# Autodesk Inventor assembly: DishBoard
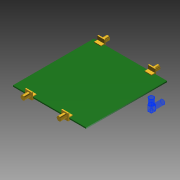
[picture p0: Inventor's stored thumbnail of the model, 180x180]
Saved by Autodesk Inventor 2014 (Build 180170000, 170)
## iProperties
Created: 2015-01-07
Part Number: DishBoard
Document SubType Name: Assembly
Designer: Owner
Author: Owner
## Documents named in this file (5)
- C:\Users\Owner\Documents\APC\FrontEnd\IAM\Dish\DishBoard.iam
- C:\Users\Owner\Documents\APC\FrontEnd\IAM\Dish\Dish_Board.ipt
- C:\Users\Owner\Documents\APC\FrontEnd\IAM\Common\SMA_Edge.ipt
- C:\Users\Owner\Documents\APC\FrontEnd\IAM\Common\SMA_Up.ipt
- C:\Users\Owner\Documents\APC\FrontEnd\IAM\Common\SMA_RightAngle.ipt
## Components (7 placed, 4 different names)
1. Dish_Board:1 — Mate:1, Mate:2, Mate:3, Mate:4, Mate:5, Mate:6, Mate:7, Mate:8, Flush:1, Flush:2, Flush:3, Flush:4, Mate:9
2. SMA_Edge:1 — Mate:5, Mate:7, Flush:1
3. SMA_Edge:2 — Mate:6, Mate:8, Flush:2
4. SMA_Edge:3 — Mate:1, Mate:2, Flush:4
5. SMA_Edge:4 — Mate:3, Mate:4, Flush:3
6. SMA_Up:1 — Mate:9, Mate:10, Mate:11
7. SMA_RightAngle:1 — Mate:10, Mate:11
## Relationships (15: Mate 11, Flush 4)
- Mate:1: Dish_Board:1 ↔ SMA_Edge:3
- Mate:2: Dish_Board:1 ↔ SMA_Edge:3
- Mate:3: Dish_Board:1 ↔ SMA_Edge:4
- Mate:4: Dish_Board:1 ↔ SMA_Edge:4
- Mate:5: Dish_Board:1 ↔ SMA_Edge:1
- Mate:6: Dish_Board:1 ↔ SMA_Edge:2
- Mate:7: Dish_Board:1 ↔ SMA_Edge:1
- Mate:8: Dish_Board:1 ↔ SMA_Edge:2
- Flush:1 (23.4442 mm): Dish_Board:1 ↔ SMA_Edge:1
- Flush:2 (-18.542 mm): Dish_Board:1 ↔ SMA_Edge:2
- Flush:3 (-17.018 mm): Dish_Board:1 ↔ SMA_Edge:4
- Flush:4 (5.08 mm): Dish_Board:1 ↔ SMA_Edge:3
- Mate:9: Dish_Board:1 ↔ SMA_Up:1
- Mate:10 (2 mm): SMA_Up:1 ↔ SMA_RightAngle:1
- Mate:11: SMA_Up:1 ↔ SMA_RightAngle:1
